# Autodesk Inventor assembly: HUB BOTTOM
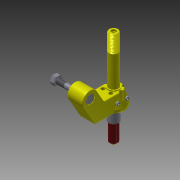
[picture p0: Inventor's stored thumbnail of the model, 180x180]
Saved by Autodesk Inventor 2013 (Build 170138000, 138)
## iProperties
Created: 2013-11-26
Part Number: HUB BOTTOM
Document SubType Name: Assembly
Designer: employee
Author: employee
## Documents named in this file (8)
- C:\Users\employee\Desktop\ConceptFORGE\ConceptFORGE\GUS Simpson\INVENTOR FILES\HUB BOTTOM.iam
- C:\Users\employee\Desktop\ConceptFORGE\ConceptFORGE\GUS Simpson\INVENTOR FILES\HUB BOTTOM.ipt
- C:\Users\employee\Desktop\ConceptFORGE\ConceptFORGE\GUS Simpson\INVENTOR FILES\M8x55.ipt
- C:\Users\employee\Desktop\ConceptFORGE\ConceptFORGE\GUS Simpson\INVENTOR FILES\M8 WASHER.ipt
- C:\Users\employee\Desktop\ConceptFORGE\ConceptFORGE\GUS Simpson\INVENTOR FILES\M8 NUT.ipt
- C:\Users\employee\Desktop\ConceptFORGE\ConceptFORGE\GUS Simpson\INVENTOR FILES\M3 NUT.ipt
- C:\Users\employee\Desktop\ConceptFORGE\ConceptFORGE\GUS Simpson\INVENTOR FILES\_UBIS.ipt
- C:\Users\employee\Desktop\ConceptFORGE\ConceptFORGE\GUS Simpson\INVENTOR FILES\M3x25.ipt
## Components (9 placed, 7 different names)
1. HUB BOTTOM:1 — Insert:1, Angle:1, Insert:2, Insert:8, Insert:9, Insert:10, Angle:2, Angle:3, Insert:11, Insert:12
2. M8x55:1 — Insert:1, Angle:1
3. M8 WASHER:1 — Insert:2, Insert:3
4. M8 NUT:1 — Insert:3
5. M3 NUT:1 — Insert:10, Angle:2
6. M3 NUT:2 — Insert:9, Angle:3
7. _UBIS:1 — Insert:8
8. M3x25:1 — Insert:11
9. M3x25:2 — Insert:12
## Relationships (11: Insert 8, Angle 3)
- Insert:1: HUB BOTTOM:1 ↔ M8x55:1
- Angle:1 (0 deg): HUB BOTTOM:1 ↔ M8x55:1
- Insert:2: HUB BOTTOM:1 ↔ M8 WASHER:1
- Insert:3 (25 mm): M8 WASHER:1 ↔ M8 NUT:1
- Insert:8: HUB BOTTOM:1 ↔ _UBIS:1
- Insert:9: HUB BOTTOM:1 ↔ M3 NUT:2
- Insert:10: HUB BOTTOM:1 ↔ M3 NUT:1
- Angle:2 (0 deg): HUB BOTTOM:1 ↔ M3 NUT:1
- Angle:3 (0 deg): HUB BOTTOM:1 ↔ M3 NUT:2
- Insert:11: HUB BOTTOM:1 ↔ M3x25:1
- Insert:12: HUB BOTTOM:1 ↔ M3x25:2
